# Autodesk Inventor assembly: ENSAMBLE_2
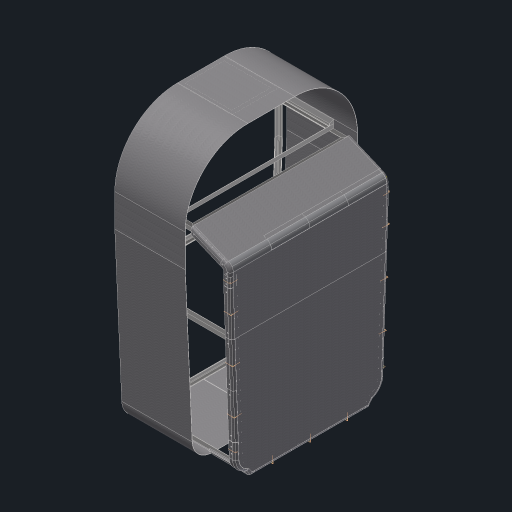
[picture p0: Inventor's stored thumbnail of the model, 512x512]
Saved by Autodesk Inventor 2024.3 (Build 283343000, 343)
## iProperties
Created: 2024-06-14
Part Number: ENSAMBLE_2
Material: Generic
Document SubType Name: Assembly
Designer: Niler
Author: Niler
## Documents named in this file (6)
- C:\Users\Niler\OneDrive\Escritorio\RECICLADOR\RECICLADOR_MODELO_3D\VERSION_3_COMPLETA\ENSAMBLE_2.iam
- C:\Users\Niler\OneDrive\Escritorio\RECICLADOR\RECICLADOR_MODELO_3D\VERSION_3_COMPLETA\CARCASA_ESTRUCTURA_Y_CHAPAS.iam
- C:\Users\Niler\OneDrive\Escritorio\RECICLADOR\RECICLADOR_MODELO_3D\VERSION_3_COMPLETA\PIEZAS_CHAPAS_ALUMINIO\CARCASA_ALUM_1.ipt
- C:\Users\Niler\OneDrive\Escritorio\RECICLADOR\RECICLADOR_MODELO_3D\VERSION_3_COMPLETA\ESQUINAS\ESQUINA_REDONDEADA_R20_P10.ipt
- C:\Users\Niler\OneDrive\Escritorio\RECICLADOR\RECICLADOR_MODELO_3D\VERSION_3_COMPLETA\ESQUINAS\ESQUINA_REDONDEADA_R20_P11.ipt
- C:\Users\Niler\OneDrive\Escritorio\RECICLADOR\RECICLADOR_MODELO_3D\VERSION_3_COMPLETA\ESQUINAS\ESQUINA_REDONDEADA_R20_P12.ipt
## Components (9 placed, 5 different names)
1. CARCASA_ESTRUCTURA_Y_CHAPAS:1 [sub-assembly] — Mate:1, Flush:1, Mate:2, Mate:3, Mate:6, Mate:13, Mate:14, Mate:15
2. CARCASA_ALUM_1:1 — Mate:1, Flush:1
3. ESQUINA_REDONDEADA_R20_P10:1 — Mate:2, Mate:4, Mate:5, Mate:6, Mate:9, Flush:2, Flush:3
4. ESQUINA_REDONDEADA_R20_P11:1 — Mate:3, Mate:4, Mate:5
5. ESQUINA_REDONDEADA_R20_P10:2 — Mate:9, Flush:2, Flush:3, Flush:4, Flush:5, Mate:12
6. ESQUINA_REDONDEADA_R20_P11:2
7. ESQUINA_REDONDEADA_R20_P10:3 — Flush:4, Flush:5, Mate:12
8. ESQUINA_REDONDEADA_R20_P11:3
9. ESQUINA_REDONDEADA_R20_P12:1 — Mate:13, Mate:14, Mate:15
## Relationships (20: Mate 15, Flush 5)
- Mate:1: CARCASA_ESTRUCTURA_Y_CHAPAS:1 ↔ CARCASA_ALUM_1:1
- Flush:1: CARCASA_ESTRUCTURA_Y_CHAPAS:1 ↔ CARCASA_ALUM_1:1
- Mate:2: CARCASA_ESTRUCTURA_Y_CHAPAS:1 ↔ ESQUINA_REDONDEADA_R20_P10:1
- Mate:3: CARCASA_ESTRUCTURA_Y_CHAPAS:1 ↔ ESQUINA_REDONDEADA_R20_P11:1
- Mate:4: ESQUINA_REDONDEADA_R20_P10:1 ↔ ESQUINA_REDONDEADA_R20_P11:1
- Mate:5: ESQUINA_REDONDEADA_R20_P10:1 ↔ ESQUINA_REDONDEADA_R20_P11:1
- Mate:6: CARCASA_ESTRUCTURA_Y_CHAPAS:1 ↔ ESQUINA_REDONDEADA_R20_P10:1
- [Mate]: ESQUINA_REDONDEADA_R20_P10:2 ↔ ESQUINA_REDONDEADA_R20_P11:2
- [Mate]: ESQUINA_REDONDEADA_R20_P10:2 ↔ ESQUINA_REDONDEADA_R20_P11:2
- Mate:9: ESQUINA_REDONDEADA_R20_P10:1 ↔ ESQUINA_REDONDEADA_R20_P10:2
- Flush:2: ESQUINA_REDONDEADA_R20_P10:1 ↔ ESQUINA_REDONDEADA_R20_P10:2
- Flush:3: ESQUINA_REDONDEADA_R20_P10:1 ↔ ESQUINA_REDONDEADA_R20_P10:2
- [Mate]: ESQUINA_REDONDEADA_R20_P10:3 ↔ ESQUINA_REDONDEADA_R20_P11:3
- [Mate]: ESQUINA_REDONDEADA_R20_P10:3 ↔ ESQUINA_REDONDEADA_R20_P11:3
- Flush:4: ESQUINA_REDONDEADA_R20_P10:2 ↔ ESQUINA_REDONDEADA_R20_P10:3
- Flush:5: ESQUINA_REDONDEADA_R20_P10:2 ↔ ESQUINA_REDONDEADA_R20_P10:3
- Mate:12: ESQUINA_REDONDEADA_R20_P10:2 ↔ ESQUINA_REDONDEADA_R20_P10:3
- Mate:13: CARCASA_ESTRUCTURA_Y_CHAPAS:1 ↔ ESQUINA_REDONDEADA_R20_P12:1
- Mate:14: CARCASA_ESTRUCTURA_Y_CHAPAS:1 ↔ ESQUINA_REDONDEADA_R20_P12:1
- Mate:15: CARCASA_ESTRUCTURA_Y_CHAPAS:1 ↔ ESQUINA_REDONDEADA_R20_P12:1
## Named parameters: d8_d4 = 0 mm, d9_d5 = 0 mm, d13_d4 = 0 mm, d14_d5 = 0 mm
